# Autodesk Inventor assembly: 足首_1_MIR
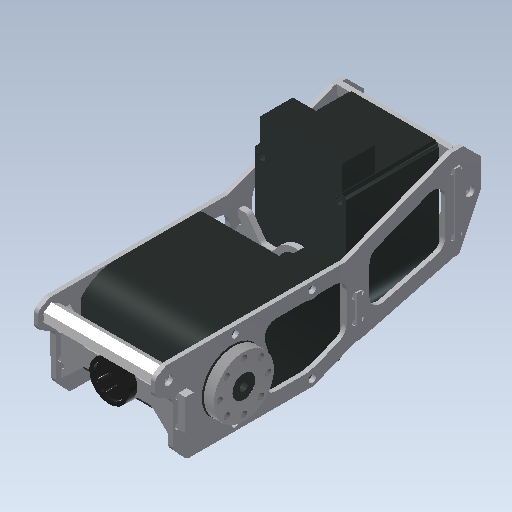
[picture p0: Inventor's stored thumbnail of the model, 512x512]
Saved by Autodesk Inventor 2020 (Build 240168000, 168)
## iProperties
Created: 2016-04-27
Part Number: 足首_1_MIR
Document SubType Name: Assembly
Designer: hiroaki
Mass: 228.077 g
Surface Area: 379.105 cm^2
Volume: 115.513 cm^3
Density: 1.97447 g/cm^3
Author: hiroaki
## Documents named in this file (11)
- C:\Users\6343y\Documents\Inventor\GankenKun\OpenPlatform_ver3_0\下半身\足首\足首_1_MIR.iam
- C:\Users\6343y\Documents\Inventor\GankenKun\OpenPlatform_ver3_0\既製品\B3M11xx.ipt
- C:\Users\6343y\Documents\Inventor\GankenKun\OpenPlatform_ver3_0\既製品\free_horn.ipt
- C:\Users\6343y\Documents\Inventor\GankenKun\OpenPlatform_ver3_0\下半身\足首\足首_メインフレーム_1_1.ipt
- C:\Users\6343y\Documents\Inventor\GankenKun\OpenPlatform_ver3_0\下半身\足首\足首_サブフレーム_1_1.ipt
- C:\Users\6343y\Documents\Inventor\GankenKun\OpenPlatform_ver3_0\下半身\足首\足首_サブフレーム_1_2.ipt
- C:\Users\6343y\Documents\Inventor\GankenKun\OpenPlatform_ver3_0\下半身\足首\足首_メインフレーム_1_1_MIR.ipt
- C:\Users\6343y\Documents\Inventor\GankenKun\OpenPlatform_ver3_0\下半身\足首\足首_サブフレーム_1_3.ipt
- C:\Users\6343y\Documents\Inventor\GankenKun\OpenPlatform_ver3_0\既製品\B3M10xx.ipt
- C:\Users\6343y\Documents\Inventor\GankenKun\OpenPlatform_ver3_0\既製品\ASU-340.ipt
- C:\Users\6343y\Documents\Inventor\GankenKun\OpenPlatform_ver3_0\下半身_160823\付け根\付け根_サブフレーム_1_4.ipt
## Components (11 placed, 9 different names)
1. B3M11xx:1 — 挿入:23, 挿入:52, 挿入:53, 挿入:54, 挿入:55, 挿入:56, 挿入:57, 挿入:58, 挿入:59
2. free_horn:1 — 挿入:23
3. 足首_メインフレーム_1_1:1 — メイト:1, メイト:2, メイト:3, メイト:4, メイト:5, メイト:6, メイト:8, 挿入:46, 挿入:48, 角度:2, 挿入:56, 挿入:57, 挿入:58, 挿入:59
4. 足首_サブフレーム_1_1:1 — メイト:1, メイト:2, メイト:3, 挿入:42, 挿入:45
5. 足首_サブフレーム_1_2:1 — メイト:4, メイト:5, メイト:6, 挿入:43, 挿入:44
6. 足首_メインフレーム_1_1_MIR:1 — メイト:9, 挿入:47, 挿入:49, 角度:1, メイト:10, 挿入:52, 挿入:53, 挿入:54, 挿入:55
7. 足首_サブフレーム_1_3:1 — メイト:8, メイト:9, メイト:10, 挿入:60
8. B3M11xx:3 — 挿入:42, 挿入:43, 挿入:44, 挿入:45
9. ASU-340:1 — 挿入:46, 挿入:47, 角度:1
10. ASU-340:2 — 挿入:48, 挿入:49, 角度:2
11. 付け根_サブフレーム_1_4:1 — 挿入:60
## Relationships (29: Insert 18, Mate 9, Angle 2)
- 挿入:23 [Insert] (0.2 mm): B3M11xx:1 ↔ free_horn:1
- メイト:1 [Mate] (0.025 mm): 足首_メインフレーム_1_1:1 ↔ 足首_サブフレーム_1_1:1
- メイト:2 [Mate]: 足首_メインフレーム_1_1:1 ↔ 足首_サブフレーム_1_1:1
- メイト:3 [Mate] (0.025 mm): 足首_メインフレーム_1_1:1 ↔ 足首_サブフレーム_1_1:1
- メイト:4 [Mate]: 足首_メインフレーム_1_1:1 ↔ 足首_サブフレーム_1_2:1
- メイト:5 [Mate] (0.025 mm): 足首_メインフレーム_1_1:1 ↔ 足首_サブフレーム_1_2:1
- メイト:6 [Mate] (0.025 mm): 足首_メインフレーム_1_1:1 ↔ 足首_サブフレーム_1_2:1
- メイト:8 [Mate]: 足首_メインフレーム_1_1:1 ↔ 足首_サブフレーム_1_3:1
- メイト:9 [Mate] (0.025 mm): 足首_メインフレーム_1_1_MIR:1 ↔ 足首_サブフレーム_1_3:1
- 挿入:42 [Insert]: 足首_サブフレーム_1_1:1 ↔ B3M11xx:3
- 挿入:43 [Insert]: 足首_サブフレーム_1_2:1 ↔ B3M11xx:3
- 挿入:44 [Insert]: 足首_サブフレーム_1_2:1 ↔ B3M11xx:3
- 挿入:45 [Insert]: 足首_サブフレーム_1_1:1 ↔ B3M11xx:3
- 挿入:46 [Insert]: 足首_メインフレーム_1_1:1 ↔ ASU-340:1
- 挿入:47 [Insert]: 足首_メインフレーム_1_1_MIR:1 ↔ ASU-340:1
- 挿入:48 [Insert]: 足首_メインフレーム_1_1:1 ↔ ASU-340:2
- 挿入:49 [Insert]: 足首_メインフレーム_1_1_MIR:1 ↔ ASU-340:2
- 角度:1 [Angle] (0 deg): 足首_メインフレーム_1_1_MIR:1 ↔ ASU-340:1
- 角度:2 [Angle] (0 deg): 足首_メインフレーム_1_1:1 ↔ ASU-340:2
- メイト:10 [Mate] (0.025 mm): 足首_メインフレーム_1_1_MIR:1 ↔ 足首_サブフレーム_1_3:1
- 挿入:52 [Insert]: B3M11xx:1 ↔ 足首_メインフレーム_1_1_MIR:1
- 挿入:53 [Insert]: B3M11xx:1 ↔ 足首_メインフレーム_1_1_MIR:1
- 挿入:54 [Insert]: B3M11xx:1 ↔ 足首_メインフレーム_1_1_MIR:1
- 挿入:55 [Insert]: B3M11xx:1 ↔ 足首_メインフレーム_1_1_MIR:1
- 挿入:56 [Insert]: B3M11xx:1 ↔ 足首_メインフレーム_1_1:1
- 挿入:57 [Insert]: B3M11xx:1 ↔ 足首_メインフレーム_1_1:1
- 挿入:58 [Insert]: B3M11xx:1 ↔ 足首_メインフレーム_1_1:1
- 挿入:59 [Insert]: B3M11xx:1 ↔ 足首_メインフレーム_1_1:1
- 挿入:60 [Insert]: 足首_サブフレーム_1_3:1 ↔ 付け根_サブフレーム_1_4:1
